# Autodesk Inventor assembly: L1 Gearbox Assembly
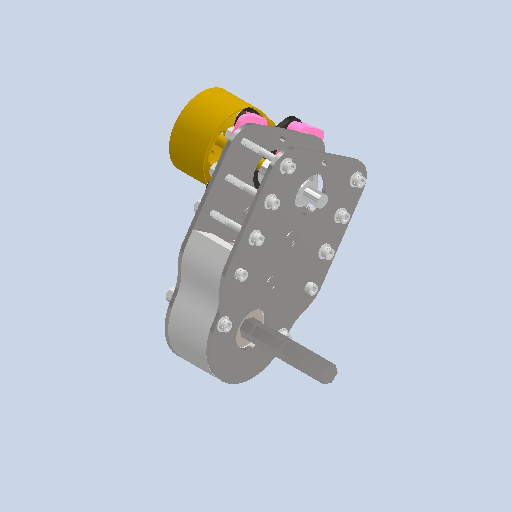
[picture p0: Inventor's stored thumbnail of the model, 512x512]
Saved by Autodesk Inventor 2025.1 (Build 291241020, 241B)
## iProperties
Created: 2023-02-14
Part Number: L1 Gearbox Assembly
Document SubType Name: Assembly
Designer: Dave
Mass: 913.46 g
Surface Area: 1660.69 cm^2
Volume: 243.163 cm^3
Density: 3.75658 g/cm^3
Author: Dave
## Documents named in this file (16)
- C:\Users\t205b\OneDrive\Documents\Github\BehrendURCMechanical\CAD\Chassis V3\CH3-L1SingleGearbox.iam
- C:\Users\t205b\OneDrive\Documents\Github\BehrendURCMechanical\CAD\Chassis V3\[Retired] GearBox\Final Gears and Assemblies\CH-1-01-20T_Drive Gear.ipt
- C:\Users\t205b\OneDrive\Documents\Github\BehrendURCMechanical\CAD\Chassis V3\[Retired] GearBox\Final Gears and Assemblies\CH-1-01-60T_Output.ipt
- C:\Users\t205b\OneDrive\Documents\Github\BehrendURCMechanical\CAD\Chassis V3\[Retired] GearBox\Final Gears and Assemblies\CH-1-01-20T_Idler.ipt
- C:\Users\t205b\OneDrive\Documents\Github\BehrendURCMechanical\CAD\Chassis V3\[Retired] GearBox\Final Gears and Assemblies\CH-1-01-60T_Idler.ipt
- C:\Users\t205b\OneDrive\Documents\Github\BehrendURCMechanical\CAD\Chassis [Retired]\GearBox\Drive Motor Shaft Coupler.ipt
- C:\Users\t205b\OneDrive\Documents\Github\BehrendURCMechanical\CAD\Chassis [Retired]\GearBox\Ch-1-01-0.5x4.5HexShaft.ipt
- C:\Users\t205b\OneDrive\Documents\Github\BehrendURCMechanical\CAD\Chassis [Retired]\GearBox\CH-1-01-0.25x1.875SmoothShaft.ipt
- C:\Users\t205b\OneDrive\Documents\Github\BehrendURCMechanical\CAD\Chassis [Retired]\GearBox\CH-1-01-0.5HexBearing.ipt
- C:\Users\t205b\OneDrive\Documents\Github\BehrendURCMechanical\CAD\Chassis [Retired]\GearBox\CH-1-01-0.25IDSmoothBoreBearing.ipt
- C:\Users\t205b\OneDrive\Documents\Github\BehrendURCMechanical\CAD\Chassis V3\DriveMotorAssem\DriveMotorAssem.iam
- C:\Users\t205b\OneDrive\Documents\Github\BehrendURCMechanical\CAD\Chassis V3\Hardware\91251A252_Black-Oxide Alloy Steel Socket Head Screw.ipt
- C:\Users\t205b\OneDrive\Documents\Github\BehrendURCMechanical\CAD\Chassis V3\Hardware\91831A011_18-8 Stainless Steel Nylon-Insert Locknut.ipt
- C:\Users\t205b\OneDrive\Documents\Github\BehrendURCMechanical\CAD\Chassis V3\Hardware\90107A011_316 Stainless Steel Washer.ipt
- C:\Users\t205b\OneDrive\Documents\Github\BehrendURCMechanical\CAD\Chassis V3\L1Plate.ipt
- C:\Users\t205b\OneDrive\Documents\Github\BehrendURCMechanical\CAD\Chassis V3\CH3-L1GearboxCover.ipt
## Components (59 placed, 15 different names)
1. CH-1-01-20T_Drive Gear:1 — Insert:16
2. CH-1-01-60T_Output:1 — Mate:17, Flush:6
3. CH-1-01-20T_Idler:1 — Mate:21, Flush:5
4. CH-1-01-60T_Idler:1 — Mate:18, Mate:19, Mate:20, Flush:5, Mate:44
5. CH-1-01-20T_Idler:2 — Mate:19, Mate:22, Flush:6, Mate:43
6. CH-1-01-60T_Idler:2 — Mate:10, Mate:11, Mate:46
7. Drive Motor Shaft Coupler:1 — Insert:16, Mate:27, Mate:31, Mate:32
8. DriveMotorAssem:1 [sub-assembly] — Mate:27, Insert:59, Insert:60, Insert:61, Insert:66, Angle:2, Insert:67, Insert:68, Insert:69
9. Ch-1-01-0.5x4.5HexShaft:1 — Mate:8, Mate:9, Flush:8, Mate:34
10. CH-1-01-0.25x1.875SmoothShaft:1 — Insert:13, Mate:45, Mate:46
11. CH-1-01-0.25x1.875SmoothShaft:2 — Insert:12, Flush:4, Mate:42, Mate:43, Mate:44
12. CH-1-01-0.5HexBearing:1 — Mate:17, Flush:8, Mate:33, Mate:34
13. CH-1-01-0.5HexBearing:2 — Mate:8, Mate:9, Mate:29, Mate:30
14. CH-1-01-0.25IDSmoothBoreBearing:1 — Insert:12, Mate:61
15. CH-1-01-0.25IDSmoothBoreBearing:2 — Insert:13, Mate:11, Mate:62
16. CH-1-01-0.25IDSmoothBoreBearing:3 — Flush:4, Mate:18, Mate:20, Mate:22
17. CH-1-01-0.25IDSmoothBoreBearing:4 — Mate:10, Mate:21
18. 91251A252_Black-Oxide Alloy Steel Socket Head Screw:1 — Insert:75, Mate:37
19. 91831A011_18-8 Stainless Steel Nylon-Insert Locknut:1 — Insert:85
20. 91251A252_Black-Oxide Alloy Steel Socket Head Screw:2 — Insert:74, Mate:36
21. 91831A011_18-8 Stainless Steel Nylon-Insert Locknut:2 — Insert:84
22. 91251A252_Black-Oxide Alloy Steel Socket Head Screw:3 — Insert:73, Mate:35
23. 91831A011_18-8 Stainless Steel Nylon-Insert Locknut:3 — Insert:83
24. 91251A252_Black-Oxide Alloy Steel Socket Head Screw:4 — Insert:76
25. 91831A011_18-8 Stainless Steel Nylon-Insert Locknut:4 — Insert:82
26. 91251A252_Black-Oxide Alloy Steel Socket Head Screw:5 — Insert:72, Mate:38
27. 91831A011_18-8 Stainless Steel Nylon-Insert Locknut:5 — Insert:80
28. 91251A252_Black-Oxide Alloy Steel Socket Head Screw:6 — Insert:71, Mate:39
29. 91831A011_18-8 Stainless Steel Nylon-Insert Locknut:6 — Insert:79
30. 91251A252_Black-Oxide Alloy Steel Socket Head Screw:7 — Insert:70, Mate:40
31. 91831A011_18-8 Stainless Steel Nylon-Insert Locknut:7 — Insert:81
32. 91251A252_Black-Oxide Alloy Steel Socket Head Screw:8 — Insert:77, Mate:41
33. 91831A011_18-8 Stainless Steel Nylon-Insert Locknut:8 — Insert:78
34. 90107A011_316 Stainless Steel Washer:1 — Insert:61, Insert:82
35. 90107A011_316 Stainless Steel Washer:2 — Insert:75, Mate:47
36. 90107A011_316 Stainless Steel Washer:3 — Insert:74, Mate:48
37. 90107A011_316 Stainless Steel Washer:4 — Insert:60, Insert:83
38. 90107A011_316 Stainless Steel Washer:5 — Insert:73, Mate:49
39. 90107A011_316 Stainless Steel Washer:6 — Insert:59, Insert:84
40. 90107A011_316 Stainless Steel Washer:7 — Insert:53, Insert:76
41. 90107A011_316 Stainless Steel Washer:8 — Insert:51, Insert:85
42. 90107A011_316 Stainless Steel Washer:9 — Insert:57, Insert:77
43. 90107A011_316 Stainless Steel Washer:10 — Insert:55, Insert:78
44. 90107A011_316 Stainless Steel Washer:11 — Insert:70, Mate:52
45. 90107A011_316 Stainless Steel Washer:12 — Insert:67, Insert:79
46. 90107A011_316 Stainless Steel Washer:13 — Insert:71, Mate:51
47. 90107A011_316 Stainless Steel Washer:14 — Insert:68, Insert:80
48. 90107A011_316 Stainless Steel Washer:15 — Insert:72, Mate:50
49. 90107A011_316 Stainless Steel Washer:16 — Insert:69, Insert:81
50. L1Plate:1 — Mate:29, Insert:53, Insert:57, Mate:32, Mate:42, Mate:45, Mate:47, Mate:48, Mate:49, Mate:50, Mate:51, Mate:52, Mate:53, Mate:55, Mate:56, Mate:57, Mate:58, Mate:59, Mate:60, Mate:61, Mate:62
51. L1Plate:2 — Mate:30, Mate:31, Insert:51, Insert:55, Insert:66, Angle:2, Mate:33, Mate:35, Mate:36, Mate:37, Mate:38, Mate:39, Mate:40, Mate:41, Mate:54, Mate:66, Mate:67
52. CH3-L1GearboxCover:1 — Mate:53, Mate:54, Mate:63, Mate:64
53. 91251A252_Black-Oxide Alloy Steel Socket Head Screw:9 — Mate:57, Mate:58, Mate:63, Mate:68, Mate:72
54. 91251A252_Black-Oxide Alloy Steel Socket Head Screw:10 — Mate:55, Mate:59, Mate:64, Mate:65, Mate:71
55. 91251A252_Black-Oxide Alloy Steel Socket Head Screw:11 — Mate:56, Mate:60
56. 90107A011_316 Stainless Steel Washer:17 — Mate:67, Mate:68, Mate:70
57. 90107A011_316 Stainless Steel Washer:18 — Mate:65, Mate:66, Mate:69
58. 91831A011_18-8 Stainless Steel Nylon-Insert Locknut:10 — Mate:70, Mate:72
59. 91831A011_18-8 Stainless Steel Nylon-Insert Locknut:11 — Mate:69, Mate:71
## Relationships (90: Mate 55, Insert 30, Flush 4, Angle 1)
- Mate:8: Ch-1-01-0.5x4.5HexShaft:1 ↔ CH-1-01-0.5HexBearing:2
- Mate:9: Ch-1-01-0.5x4.5HexShaft:1 ↔ CH-1-01-0.5HexBearing:2
- Insert:12: CH-1-01-0.25x1.875SmoothShaft:2 ↔ CH-1-01-0.25IDSmoothBoreBearing:1
- Insert:13: CH-1-01-0.25x1.875SmoothShaft:1 ↔ CH-1-01-0.25IDSmoothBoreBearing:2
- Mate:10: CH-1-01-60T_Idler:2 ↔ CH-1-01-0.25IDSmoothBoreBearing:4
- Mate:11: CH-1-01-60T_Idler:2 ↔ CH-1-01-0.25IDSmoothBoreBearing:2
- Flush:4: CH-1-01-0.25x1.875SmoothShaft:2 ↔ CH-1-01-0.25IDSmoothBoreBearing:3
- Mate:17: CH-1-01-60T_Output:1 ↔ CH-1-01-0.5HexBearing:1
- Mate:18: CH-1-01-60T_Idler:1 ↔ CH-1-01-0.25IDSmoothBoreBearing:3
- Mate:19: CH-1-01-60T_Idler:1 ↔ CH-1-01-20T_Idler:2
- Mate:20: CH-1-01-60T_Idler:1 ↔ CH-1-01-0.25IDSmoothBoreBearing:3
- Mate:21: CH-1-01-20T_Idler:1 ↔ CH-1-01-0.25IDSmoothBoreBearing:4
- Flush:5: CH-1-01-20T_Idler:1 ↔ CH-1-01-60T_Idler:1
- Mate:22: CH-1-01-20T_Idler:2 ↔ CH-1-01-0.25IDSmoothBoreBearing:3
- Flush:6: CH-1-01-60T_Output:1 ↔ CH-1-01-20T_Idler:2
- Flush:8: Ch-1-01-0.5x4.5HexShaft:1 ↔ CH-1-01-0.5HexBearing:1
- Insert:16: CH-1-01-20T_Drive Gear:1 ↔ Drive Motor Shaft Coupler:1
- Mate:27: Drive Motor Shaft Coupler:1 ↔ DriveMotorAssem:1
- Mate:29: CH-1-01-0.5HexBearing:2 ↔ L1Plate:1
- Mate:30: CH-1-01-0.5HexBearing:2 ↔ L1Plate:2
- Mate:31: Drive Motor Shaft Coupler:1 ↔ L1Plate:2
- Insert:51: 90107A011_316 Stainless Steel Washer:8 ↔ L1Plate:2
- Insert:53: 90107A011_316 Stainless Steel Washer:7 ↔ L1Plate:1
- Insert:55: 90107A011_316 Stainless Steel Washer:10 ↔ L1Plate:2
- Insert:57: 90107A011_316 Stainless Steel Washer:9 ↔ L1Plate:1
- Insert:59: DriveMotorAssem:1 ↔ 90107A011_316 Stainless Steel Washer:6
- Insert:60: DriveMotorAssem:1 ↔ 90107A011_316 Stainless Steel Washer:4
- Insert:61: DriveMotorAssem:1 ↔ 90107A011_316 Stainless Steel Washer:1
- Insert:66: DriveMotorAssem:1 ↔ L1Plate:2
- Angle:2 (0 deg): DriveMotorAssem:1 ↔ L1Plate:2
- Insert:67: DriveMotorAssem:1 ↔ 90107A011_316 Stainless Steel Washer:12
- Insert:68: DriveMotorAssem:1 ↔ 90107A011_316 Stainless Steel Washer:14
- Insert:69: DriveMotorAssem:1 ↔ 90107A011_316 Stainless Steel Washer:16
- Mate:32: Drive Motor Shaft Coupler:1 ↔ L1Plate:1
- Insert:70: 91251A252_Black-Oxide Alloy Steel Socket Head Screw:7 ↔ 90107A011_316 Stainless Steel Washer:11
- Insert:71: 91251A252_Black-Oxide Alloy Steel Socket Head Screw:6 ↔ 90107A011_316 Stainless Steel Washer:13
- Insert:72: 91251A252_Black-Oxide Alloy Steel Socket Head Screw:5 ↔ 90107A011_316 Stainless Steel Washer:15
- Insert:73: 91251A252_Black-Oxide Alloy Steel Socket Head Screw:3 ↔ 90107A011_316 Stainless Steel Washer:5
- Insert:74: 91251A252_Black-Oxide Alloy Steel Socket Head Screw:2 ↔ 90107A011_316 Stainless Steel Washer:3
- Insert:75: 91251A252_Black-Oxide Alloy Steel Socket Head Screw:1 ↔ 90107A011_316 Stainless Steel Washer:2
- Insert:76: 91251A252_Black-Oxide Alloy Steel Socket Head Screw:4 ↔ 90107A011_316 Stainless Steel Washer:7
- Insert:77: 91251A252_Black-Oxide Alloy Steel Socket Head Screw:8 ↔ 90107A011_316 Stainless Steel Washer:9
- Insert:78: 91831A011_18-8 Stainless Steel Nylon-Insert Locknut:8 ↔ 90107A011_316 Stainless Steel Washer:10
- Insert:79: 91831A011_18-8 Stainless Steel Nylon-Insert Locknut:6 ↔ 90107A011_316 Stainless Steel Washer:12
- Insert:80: 91831A011_18-8 Stainless Steel Nylon-Insert Locknut:5 ↔ 90107A011_316 Stainless Steel Washer:14
- Insert:81: 91831A011_18-8 Stainless Steel Nylon-Insert Locknut:7 ↔ 90107A011_316 Stainless Steel Washer:16
- Insert:82: 91831A011_18-8 Stainless Steel Nylon-Insert Locknut:4 ↔ 90107A011_316 Stainless Steel Washer:1
- Insert:83: 91831A011_18-8 Stainless Steel Nylon-Insert Locknut:3 ↔ 90107A011_316 Stainless Steel Washer:4
- Insert:84: 91831A011_18-8 Stainless Steel Nylon-Insert Locknut:2 ↔ 90107A011_316 Stainless Steel Washer:6
- Insert:85: 91831A011_18-8 Stainless Steel Nylon-Insert Locknut:1 ↔ 90107A011_316 Stainless Steel Washer:8
- Mate:33: CH-1-01-0.5HexBearing:1 ↔ L1Plate:2
- Mate:34: Ch-1-01-0.5x4.5HexShaft:1 ↔ CH-1-01-0.5HexBearing:1
- Mate:35: 91251A252_Black-Oxide Alloy Steel Socket Head Screw:3 ↔ L1Plate:2
- Mate:36: 91251A252_Black-Oxide Alloy Steel Socket Head Screw:2 ↔ L1Plate:2
- Mate:37: 91251A252_Black-Oxide Alloy Steel Socket Head Screw:1 ↔ L1Plate:2
- Mate:38: 91251A252_Black-Oxide Alloy Steel Socket Head Screw:5 ↔ L1Plate:2
- Mate:39: 91251A252_Black-Oxide Alloy Steel Socket Head Screw:6 ↔ L1Plate:2
- Mate:40: 91251A252_Black-Oxide Alloy Steel Socket Head Screw:7 ↔ L1Plate:2
- Mate:41: 91251A252_Black-Oxide Alloy Steel Socket Head Screw:8 ↔ L1Plate:2
- Mate:42: CH-1-01-0.25x1.875SmoothShaft:2 ↔ L1Plate:1
- Mate:43: CH-1-01-20T_Idler:2 ↔ CH-1-01-0.25x1.875SmoothShaft:2
- Mate:44: CH-1-01-60T_Idler:1 ↔ CH-1-01-0.25x1.875SmoothShaft:2
- Mate:45: CH-1-01-0.25x1.875SmoothShaft:1 ↔ L1Plate:1
- Mate:46: CH-1-01-60T_Idler:2 ↔ CH-1-01-0.25x1.875SmoothShaft:1
- Mate:47: 90107A011_316 Stainless Steel Washer:2 ↔ L1Plate:1
- Mate:48: 90107A011_316 Stainless Steel Washer:3 ↔ L1Plate:1
- Mate:49: 90107A011_316 Stainless Steel Washer:5 ↔ L1Plate:1
- Mate:50: 90107A011_316 Stainless Steel Washer:15 ↔ L1Plate:1
- Mate:51: 90107A011_316 Stainless Steel Washer:13 ↔ L1Plate:1
- Mate:52: 90107A011_316 Stainless Steel Washer:11 ↔ L1Plate:1
- Mate:53: L1Plate:1 ↔ CH3-L1GearboxCover:1
- Mate:54: L1Plate:2 ↔ CH3-L1GearboxCover:1
- Mate:55: L1Plate:1 ↔ 91251A252_Black-Oxide Alloy Steel Socket Head Screw:10
- Mate:56: L1Plate:1 ↔ 91251A252_Black-Oxide Alloy Steel Socket Head Screw:11
- Mate:57: L1Plate:1 ↔ 91251A252_Black-Oxide Alloy Steel Socket Head Screw:9
- Mate:58: L1Plate:1 ↔ 91251A252_Black-Oxide Alloy Steel Socket Head Screw:9
- Mate:59: L1Plate:1 ↔ 91251A252_Black-Oxide Alloy Steel Socket Head Screw:10
- Mate:60: L1Plate:1 ↔ 91251A252_Black-Oxide Alloy Steel Socket Head Screw:11
- Mate:61: CH-1-01-0.25IDSmoothBoreBearing:1 ↔ L1Plate:1
- Mate:62: CH-1-01-0.25IDSmoothBoreBearing:2 ↔ L1Plate:1
- Mate:63: CH3-L1GearboxCover:1 ↔ 91251A252_Black-Oxide Alloy Steel Socket Head Screw:9
- Mate:64: CH3-L1GearboxCover:1 ↔ 91251A252_Black-Oxide Alloy Steel Socket Head Screw:10
- Mate:65: 91251A252_Black-Oxide Alloy Steel Socket Head Screw:10 ↔ 90107A011_316 Stainless Steel Washer:18
- Mate:66: L1Plate:2 ↔ 90107A011_316 Stainless Steel Washer:18
- Mate:67: L1Plate:2 ↔ 90107A011_316 Stainless Steel Washer:17
- Mate:68: 91251A252_Black-Oxide Alloy Steel Socket Head Screw:9 ↔ 90107A011_316 Stainless Steel Washer:17
- Mate:69: 90107A011_316 Stainless Steel Washer:18 ↔ 91831A011_18-8 Stainless Steel Nylon-Insert Locknut:11
- Mate:70: 90107A011_316 Stainless Steel Washer:17 ↔ 91831A011_18-8 Stainless Steel Nylon-Insert Locknut:10
- Mate:71: 91251A252_Black-Oxide Alloy Steel Socket Head Screw:10 ↔ 91831A011_18-8 Stainless Steel Nylon-Insert Locknut:11
- Mate:72: 91251A252_Black-Oxide Alloy Steel Socket Head Screw:9 ↔ 91831A011_18-8 Stainless Steel Nylon-Insert Locknut:10
